# Autodesk Inventor assembly: claws_endeffector_8_5_rotary-blade
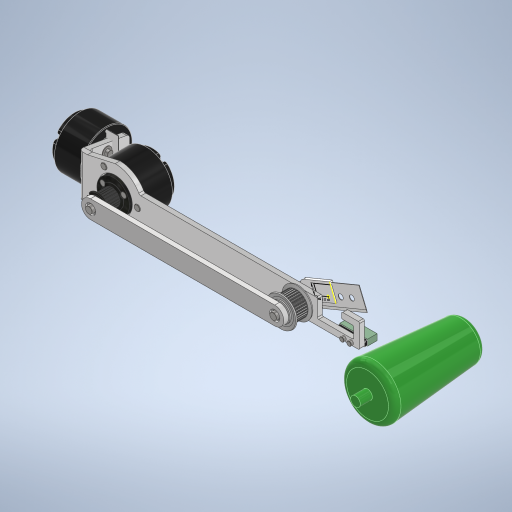
[picture p0: Inventor's stored thumbnail of the model, 512x512]
Saved by Autodesk Inventor 2024 (Build 280153000, 153)
## iProperties
Created: 2025-06-01
Part Number: claws_endeffector_8_5_rotary-blade
Document SubType Name: Assembly
Designer: 1412z
Author: 1412z
## Documents named in this file (22)
- C:\Users\1412z\OneDrive\デスクトップ\rdclab\harvesting_robot\harvesting_endeffector\claws_endeffector\claws_endeffector_8_5_rotary-blade.iam
- C:\Users\1412z\OneDrive\デスクトップ\rdclab\harvesting_robot\harvesting_endeffector\claws_endeffector\motor_holder\motor_holder_8-5.ipt
- C:\Users\1412z\OneDrive\デスクトップ\rdclab\harvesting_robot\harvesting_endeffector\claws_endeffector\GIM3505-08\GIM3505-8_with-driver.ipt
- C:\Users\1412z\OneDrive\デスクトップ\rdclab\harvesting_robot\harvesting_endeffector\claws_endeffector\misumi\washer\washer_M3.ipt
- C:\Users\1412z\OneDrive\デスクトップ\rdclab\harvesting_robot\harvesting_endeffector\claws_endeffector\misumi\M2.5×4\M2.5×4.ipt
- C:\Users\1412z\OneDrive\デスクトップ\rdclab\harvesting_robot\harvesting_endeffector\claws_endeffector\misumi\HTPA22S2M100-A-V4-Z6-J3_Autodesk_Inventor_2024_20250304\HTPA22S2M100-A-V4-Z6-J3_0_a-3.ipt
- C:\Users\1412z\OneDrive\デスクトップ\rdclab\harvesting_robot\harvesting_endeffector\claws_endeffector\misumi\SFL674ZZ_Autodesk_Inventor_2024_20250304\SFL674ZZ.ipt
- C:\Users\1412z\OneDrive\デスクトップ\rdclab\harvesting_robot\harvesting_endeffector\claws_endeffector\misumi\simring\simring_Φ4-Φ5.ipt
- C:\Users\1412z\OneDrive\デスクトップ\rdclab\harvesting_robot\harvesting_endeffector\claws_endeffector\misumi\HTPA32S2M100-A-P4_Autodesk_Inventor_2024_20250404\AIS2024\HTPA32S2M100-A-P4_a.ipt
- C:\Users\1412z\OneDrive\デスクトップ\rdclab\harvesting_robot\harvesting_endeffector\claws_endeffector\misumi\washer\washer_M4.ipt
- C:\Users\1412z\OneDrive\デスクトップ\rdclab\harvesting_robot\harvesting_endeffector\claws_endeffector\motor_holder\motor_holder_top_2.ipt
- C:\Users\1412z\OneDrive\デスクトップ\rdclab\harvesting_robot\harvesting_endeffector\claws_endeffector\misumi\shaft\shaft_31.7mm_Dcut.ipt
- C:\Users\1412z\OneDrive\デスクトップ\rdclab\harvesting_robot\harvesting_endeffector\claws_endeffector\misumi\shaft\shaft_15.05.ipt
- C:\Users\1412z\OneDrive\デスクトップ\rdclab\harvesting_robot\harvesting_endeffector\claws_endeffector\misumi\M3×8\M3×8.ipt
- C:\Users\1412z\OneDrive\デスクトップ\rdclab\harvesting_robot\harvesting_endeffector\claws_endeffector\misumi\M3×4\M3×4.ipt
- C:\Users\1412z\OneDrive\デスクトップ\rdclab\harvesting_robot\harvesting_endeffector\claws_endeffector\cutter_part\cutter_XB210.ipt
- C:\Users\1412z\OneDrive\デスクトップ\rdclab\harvesting_robot\harvesting_endeffector\Vibrating_knife_endeffector\model\green_pepper_model.ipt
- C:\Users\1412z\OneDrive\デスクトップ\rdclab\harvesting_robot\harvesting_endeffector\claws_endeffector\misumi\M2×6\M2×6.ipt
- C:\Users\1412z\OneDrive\デスクトップ\rdclab\harvesting_robot\harvesting_endeffector\claws_endeffector\cutter_part\cutter_board_claws_endeffector_8_5_rotary-blade-2.ipt
- C:\Users\1412z\OneDrive\デスクトップ\rdclab\harvesting_robot\harvesting_endeffector\claws_endeffector\cutter_part\cutter_stopper.ipt
- C:\Users\1412z\OneDrive\デスクトップ\rdclab\harvesting_robot\harvesting_endeffector\claws_endeffector\cutter_part\griper_TPU-2.ipt
- C:\Users\1412z\OneDrive\デスクトップ\rdclab\harvesting_robot\harvesting_endeffector\claws_endeffector\misumi\M2×8\M2×8.ipt
## Components (42 placed, 21 different names)
1. motor_holder_8-5:1 — 回転:1, 回転:2, 回転:3, 回転:4, 回転:5, 回転:6, 回転:7, 回転:11, 回転:12, 回転:13, 回転:19, 回転:20, 回転:54, 回転:55, 回転:62, 回転:63
2. GIM3505-8_with-driver:1 — 回転:1, 回転:2, 回転:14, 回転:15
3. GIM3505-8_with-driver:2 — 回転:3, 回転:4
4. washer_M3:1 — 回転:7, 回転:10
5. washer_M3:2 — 回転:6, 回転:9
6. washer_M3:3 — 回転:5, 回転:8
7. M2.5×4:1 — 回転:10
8. M2.5×4:2 — 回転:9
9. M2.5×4:3 — 回転:8
10. M2.5×4:4 — 回転:11
11. M2.5×4:5 — 回転:12
12. M2.5×4:6 — 回転:13
13. HTPA22S2M100-A-V4-Z6-J3_0_a-3:1 — 回転:14, 回転:15, 回転:16, 回転:17, 回転:18, 回転:25, 回転:31
14. M2.5×4:7 — 回転:18
15. M2.5×4:8 — 回転:16
16. M2.5×4:9 — 回転:17
17. SFL674ZZ:1 — 回転:19, 回転:21
18. SFL674ZZ:2 — 回転:20, 回転:22
19. simring_Φ4-Φ5:1 — 回転:22, 回転:23
20. simring_Φ4-Φ5:2 — 回転:21, 回転:46
21. HTPA32S2M100-A-P4_a:1 — 回転:23, 回転:24
22. washer_M4:1 — 回転:24, 回転:26
23. washer_M4:2 — 回転:25, 回転:27
24. motor_holder_top_2:1 — 回転:26, 回転:27, 回転:28, 回転:29
25. SFL674ZZ:3 — 回転:28, 回転:30
26. SFL674ZZ:4 — 回転:29, 回転:32
27. shaft_31.7mm_Dcut:1 — 回転:30, 回転:35
28. shaft_15.05:1 — 回転:32, 回転:34
29. washer_M4:3 — 回転:31, 回転:33
30. M3×8:1 — 回転:33
31. M3×4:1 — 回転:34
32. M3×4:2 — 回転:35
33. green_pepper_model:1
34. cutter_board_claws_endeffector_8_5_rotary-blade-2:1 — 回転:46, 回転:68
35. M2×6:3 — 回転:54
36. M2×6:4 — 回転:55
37. cutter_stopper:1 — 回転:62, 回転:63, 回転:64, 回転:65
38. griper_TPU-2:1 — 回転:64, 回転:65, 回転:66, 回転:67
39. M2×8:1 — 回転:66
40. M2×8:2 — 回転:67
41. cutter_XB210:1
42. cutter_XB210:2 — 回転:68
## Relationships (45: RevoluteJoint 45)
- 回転:1 [RevoluteJoint]: motor_holder_8-5:1 ↔ GIM3505-8_with-driver:1
- 回転:2 [RevoluteJoint]: motor_holder_8-5:1 ↔ GIM3505-8_with-driver:1
- 回転:3 [RevoluteJoint]: motor_holder_8-5:1 ↔ GIM3505-8_with-driver:2
- 回転:4 [RevoluteJoint]: motor_holder_8-5:1 ↔ GIM3505-8_with-driver:2
- 回転:5 [RevoluteJoint]: motor_holder_8-5:1 ↔ washer_M3:3
- 回転:6 [RevoluteJoint]: motor_holder_8-5:1 ↔ washer_M3:2
- 回転:7 [RevoluteJoint]: motor_holder_8-5:1 ↔ washer_M3:1
- 回転:8 [RevoluteJoint]: washer_M3:3 ↔ M2.5×4:3
- 回転:9 [RevoluteJoint]: washer_M3:2 ↔ M2.5×4:2
- 回転:10 [RevoluteJoint]: washer_M3:1 ↔ M2.5×4:1
- 回転:11 [RevoluteJoint]: motor_holder_8-5:1 ↔ M2.5×4:4
- 回転:12 [RevoluteJoint]: motor_holder_8-5:1 ↔ M2.5×4:5
- 回転:13 [RevoluteJoint]: motor_holder_8-5:1 ↔ M2.5×4:6
- 回転:14 [RevoluteJoint]: GIM3505-8_with-driver:1 ↔ HTPA22S2M100-A-V4-Z6-J3_0_a-3:1
- 回転:15 [RevoluteJoint]: GIM3505-8_with-driver:1 ↔ HTPA22S2M100-A-V4-Z6-J3_0_a-3:1
- 回転:16 [RevoluteJoint]: HTPA22S2M100-A-V4-Z6-J3_0_a-3:1 ↔ M2.5×4:8
- 回転:17 [RevoluteJoint]: HTPA22S2M100-A-V4-Z6-J3_0_a-3:1 ↔ M2.5×4:9
- 回転:18 [RevoluteJoint]: HTPA22S2M100-A-V4-Z6-J3_0_a-3:1 ↔ M2.5×4:7
- 回転:19 [RevoluteJoint]: motor_holder_8-5:1 ↔ SFL674ZZ:1
- 回転:20 [RevoluteJoint]: motor_holder_8-5:1 ↔ SFL674ZZ:2
- 回転:21 [RevoluteJoint]: SFL674ZZ:1 ↔ simring_Φ4-Φ5:2
- 回転:22 [RevoluteJoint]: SFL674ZZ:2 ↔ simring_Φ4-Φ5:1
- 回転:23 [RevoluteJoint]: simring_Φ4-Φ5:1 ↔ HTPA32S2M100-A-P4_a:1
- 回転:24 [RevoluteJoint]: HTPA32S2M100-A-P4_a:1 ↔ washer_M4:1
- 回転:25 [RevoluteJoint]: HTPA22S2M100-A-V4-Z6-J3_0_a-3:1 ↔ washer_M4:2
- 回転:26 [RevoluteJoint]: washer_M4:1 ↔ motor_holder_top_2:1
- 回転:27 [RevoluteJoint]: washer_M4:2 ↔ motor_holder_top_2:1
- 回転:28 [RevoluteJoint]: motor_holder_top_2:1 ↔ SFL674ZZ:3
- 回転:29 [RevoluteJoint]: motor_holder_top_2:1 ↔ SFL674ZZ:4
- 回転:30 [RevoluteJoint]: SFL674ZZ:3 ↔ shaft_31.7mm_Dcut:1
- 回転:31 [RevoluteJoint]: HTPA22S2M100-A-V4-Z6-J3_0_a-3:1 ↔ washer_M4:3
- 回転:32 [RevoluteJoint]: SFL674ZZ:4 ↔ shaft_15.05:1
- 回転:33 [RevoluteJoint]: washer_M4:3 ↔ M3×8:1
- 回転:34 [RevoluteJoint]: shaft_15.05:1 ↔ M3×4:1
- 回転:35 [RevoluteJoint]: shaft_31.7mm_Dcut:1 ↔ M3×4:2
- 回転:46 [RevoluteJoint]: simring_Φ4-Φ5:2 ↔ cutter_board_claws_endeffector_8_5_rotary-blade-2:1
- 回転:54 [RevoluteJoint]: motor_holder_8-5:1 ↔ M2×6:3
- 回転:55 [RevoluteJoint]: motor_holder_8-5:1 ↔ M2×6:4
- 回転:62 [RevoluteJoint]: motor_holder_8-5:1 ↔ cutter_stopper:1
- 回転:63 [RevoluteJoint]: motor_holder_8-5:1 ↔ cutter_stopper:1
- 回転:64 [RevoluteJoint]: cutter_stopper:1 ↔ griper_TPU-2:1
- 回転:65 [RevoluteJoint]: cutter_stopper:1 ↔ griper_TPU-2:1
- 回転:66 [RevoluteJoint]: griper_TPU-2:1 ↔ M2×8:1
- 回転:67 [RevoluteJoint]: griper_TPU-2:1 ↔ M2×8:2
- 回転:68 [RevoluteJoint]: cutter_board_claws_endeffector_8_5_rotary-blade-2:1 ↔ cutter_XB210:2
